# Autodesk Inventor assembly: Pnematic Screw 1764
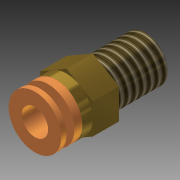
[picture p0: Inventor's stored thumbnail of the model, 180x180]
Saved by Autodesk Inventor 2011 (Build 150239000, 239)
## iProperties
Created: 2010-02-09
Part Number: Pnematic Screw 1764
Document SubType Name: Assembly
Designer: clee1
Author: clee1
## Documents named in this file (3)
- R:\CAD Archives\Pnewmatics\pnewmatic screw\Pnematic Screw 1764.iam
- R:\CAD Archives\Pnewmatics\pnewmatic screw\Pnewmatic Screw Part 1 1764.ipt
- R:\CAD Archives\Pnewmatics\pnewmatic screw\Pnewmatic Screw Part 2 1764.ipt
## Components (2 placed, 2 different names)
1. Pnewmatic Screw Part 1 1764:1 — Insert:1
2. Pnewmatic Screw Part 2 1764:1 — Insert:1
## Relationships (1: Insert 1)
- Insert:1: Pnewmatic Screw Part 1 1764:1 ↔ Pnewmatic Screw Part 2 1764:1
